# Autodesk Inventor assembly: Shipping goods colors subassembly FINAL VERSION
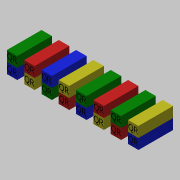
[picture p0: Inventor's stored thumbnail of the model, 180x180]
Saved by Autodesk Inventor 2015 (Build 190159000, 159)
## iProperties
Created: 2015-03-08
Part Number: Shipping goods colors subassembly FINAL VERSION
Document SubType Name: Assembly
Designer: Vukica
Author: Vukica
## Documents named in this file (5)
- D:\Dropbox\Dropbox\Service\IEEE\!Final Rules\2016Hardware_Court_v8-aug12\Shipping goods colors subassembly.iam
- D:\Dropbox\Dropbox\Service\IEEE\!Final Rules\2016Hardware_Court_v8-aug12\Container 2 2 5 colored color 2.ipt
- D:\Dropbox\Dropbox\Service\IEEE\!Final Rules\2016Hardware_Court_v8-aug12\Container 2 2 5 colored color 3.ipt
- D:\Dropbox\Dropbox\Service\IEEE\!Final Rules\2016Hardware_Court_v8-aug12\Container 2 2 5 colored color 4.ipt
- D:\Dropbox\Dropbox\Service\IEEE\!Final Rules\2016Hardware_Court_v8-aug12\Container 2 2 5 colored color 1.ipt
## Components (16 placed, 4 different names)
1. Container 2 2 5 colored color 2:1 — Mate:1, Flush:1, Flush:2, Mate:2, Flush:3, Flush:4, Flush:13, Flush:14
2. Container 2 2 5 colored color 3:1 — Mate:2, Flush:3, Flush:4, Mate:3, Flush:5, Flush:6, Mate:7
3. Container 2 2 5 colored color 4:1 — Mate:1, Flush:1, Flush:2, Mate:11, Flush:21, Flush:22
4. Container 2 2 5 colored color 1:1 — Mate:3, Flush:5, Flush:6
5. Container 2 2 5 colored color 2:2
6. Container 2 2 5 colored color 3:2
7. Container 2 2 5 colored color 4:2 — Flush:25, Mate:13, Flush:26
8. Container 2 2 5 colored color 1:2 — Mate:7, Flush:13, Flush:14, Mate:8, Flush:15, Flush:16
9. Container 2 2 5 colored color 4:3 — Mate:8, Flush:15, Flush:16, Mate:9, Flush:17, Flush:18
10. Container 2 2 5 colored color 2:3 — Mate:9, Flush:17, Flush:18
11. Container 2 2 5 colored color 3:3
12. Container 2 2 5 colored color 1:3 — Mate:11, Flush:21, Flush:22
13. Container 2 2 5 colored color 4:4 — Mate:12, Flush:23, Flush:24
14. Container 2 2 5 colored color 3:4 — Mate:14, Flush:27, Flush:28, Flush:29, Flush:30, Mate:15
15. Container 2 2 5 colored color 2:4 — Mate:12, Flush:23, Flush:24, Flush:25, Mate:13, Flush:26, Flush:29, Flush:30, Mate:15
16. Container 2 2 5 colored color 1:4 — Mate:14, Flush:27, Flush:28
## Relationships (45: Flush 30, Mate 15)
- Mate:1 (25.4 mm): Container 2 2 5 colored color 2:1 ↔ Container 2 2 5 colored color 4:1
- Flush:1: Container 2 2 5 colored color 2:1 ↔ Container 2 2 5 colored color 4:1
- Flush:2: Container 2 2 5 colored color 2:1 ↔ Container 2 2 5 colored color 4:1
- Mate:2 (25.4 mm): Container 2 2 5 colored color 2:1 ↔ Container 2 2 5 colored color 3:1
- Flush:3: Container 2 2 5 colored color 2:1 ↔ Container 2 2 5 colored color 3:1
- Flush:4: Container 2 2 5 colored color 2:1 ↔ Container 2 2 5 colored color 3:1
- Mate:3 (25.4 mm): Container 2 2 5 colored color 3:1 ↔ Container 2 2 5 colored color 1:1
- Flush:5: Container 2 2 5 colored color 3:1 ↔ Container 2 2 5 colored color 1:1
- Flush:6: Container 2 2 5 colored color 3:1 ↔ Container 2 2 5 colored color 1:1
- [Mate] (25.4 mm): Container 2 2 5 colored color 2:2 ↔ Container 2 2 5 colored color 4:2
- [Flush]: Container 2 2 5 colored color 2:2 ↔ Container 2 2 5 colored color 4:2
- [Flush]: Container 2 2 5 colored color 2:2 ↔ Container 2 2 5 colored color 4:2
- [Mate] (25.4 mm): Container 2 2 5 colored color 2:2 ↔ Container 2 2 5 colored color 3:2
- [Flush]: Container 2 2 5 colored color 2:2 ↔ Container 2 2 5 colored color 3:2
- [Flush]: Container 2 2 5 colored color 2:2 ↔ Container 2 2 5 colored color 3:2
- [Mate] (25.4 mm): Container 2 2 5 colored color 3:2 ↔ Container 2 2 5 colored color 1:2
- [Flush]: Container 2 2 5 colored color 3:2 ↔ Container 2 2 5 colored color 1:2
- [Flush]: Container 2 2 5 colored color 3:2 ↔ Container 2 2 5 colored color 1:2
- Mate:7: Container 2 2 5 colored color 3:1 ↔ Container 2 2 5 colored color 1:2
- Flush:13: Container 2 2 5 colored color 2:1 ↔ Container 2 2 5 colored color 1:2
- Flush:14: Container 2 2 5 colored color 2:1 ↔ Container 2 2 5 colored color 1:2
- Mate:8 (25.4 mm): Container 2 2 5 colored color 1:2 ↔ Container 2 2 5 colored color 4:3
- Flush:15: Container 2 2 5 colored color 1:2 ↔ Container 2 2 5 colored color 4:3
- Flush:16: Container 2 2 5 colored color 1:2 ↔ Container 2 2 5 colored color 4:3
- Mate:9 (25.4 mm): Container 2 2 5 colored color 4:3 ↔ Container 2 2 5 colored color 2:3
- Flush:17: Container 2 2 5 colored color 4:3 ↔ Container 2 2 5 colored color 2:3
- Flush:18: Container 2 2 5 colored color 4:3 ↔ Container 2 2 5 colored color 2:3
- [Mate] (25.4 mm): Container 2 2 5 colored color 3:3 ↔ Container 2 2 5 colored color 1:3
- [Flush]: Container 2 2 5 colored color 3:3 ↔ Container 2 2 5 colored color 1:3
- [Flush]: Container 2 2 5 colored color 3:3 ↔ Container 2 2 5 colored color 1:3
- Mate:11 (25.4 mm): Container 2 2 5 colored color 4:1 ↔ Container 2 2 5 colored color 1:3
- Flush:21: Container 2 2 5 colored color 4:1 ↔ Container 2 2 5 colored color 1:3
- Flush:22: Container 2 2 5 colored color 4:1 ↔ Container 2 2 5 colored color 1:3
- Mate:12: Container 2 2 5 colored color 4:4 ↔ Container 2 2 5 colored color 2:4
- Flush:23: Container 2 2 5 colored color 4:4 ↔ Container 2 2 5 colored color 2:4
- Flush:24: Container 2 2 5 colored color 4:4 ↔ Container 2 2 5 colored color 2:4
- Flush:25: Container 2 2 5 colored color 4:2 ↔ Container 2 2 5 colored color 2:4
- Mate:13 (25.4 mm): Container 2 2 5 colored color 4:2 ↔ Container 2 2 5 colored color 2:4
- Flush:26: Container 2 2 5 colored color 4:2 ↔ Container 2 2 5 colored color 2:4
- Mate:14: Container 2 2 5 colored color 3:4 ↔ Container 2 2 5 colored color 1:4
- Flush:27: Container 2 2 5 colored color 3:4 ↔ Container 2 2 5 colored color 1:4
- Flush:28: Container 2 2 5 colored color 3:4 ↔ Container 2 2 5 colored color 1:4
- Flush:29: Container 2 2 5 colored color 3:4 ↔ Container 2 2 5 colored color 2:4
- Flush:30: Container 2 2 5 colored color 3:4 ↔ Container 2 2 5 colored color 2:4
- Mate:15 (25.4 mm): Container 2 2 5 colored color 3:4 ↔ Container 2 2 5 colored color 2:4
## Named parameters: d9_d1 = 0 mm, d10_d2 = 0 mm, d11_d3 = 25.4 mm, d12_d4 = 0 mm, d13_d5 = 0 mm, d14_d6 = 25.4 mm, d15_d7 = 0 mm, d16_d8 = 0 mm, d17_d0 = 25.4 mm, d27_d6 = 25.4 mm, d28_d7 = 0 mm, d29_d8 = 0 mm
